# Autodesk Inventor assembly: Assembly1
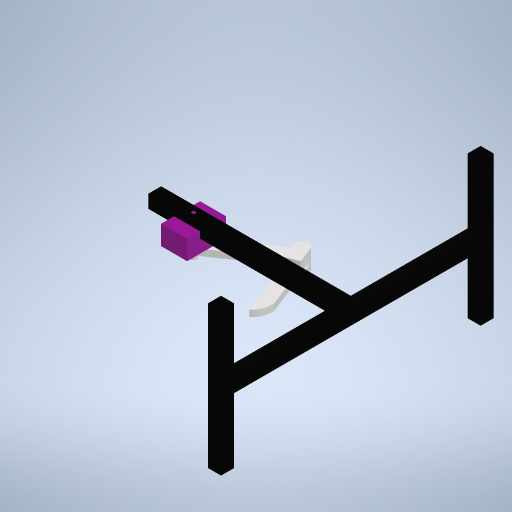
[picture p0: Inventor's stored thumbnail of the model, 512x512]
Saved by Autodesk Inventor 2024 (Build 280153000, 153)
## iProperties
Created: 2024-08-23
Part Number: Assembly1
Document SubType Name: Assembly
Designer: domko
Author: domko
## Documents named in this file (6)
- C:\Users\Public\Documents\Autodesk\Inventor 2024\czlapczlap_Leg\Assembly1.iam
- C:\Users\Public\Documents\Autodesk\Inventor 2024\czlapczlap_Leg\statyw.ipt
- C:\Users\Public\Documents\Autodesk\Inventor 2024\czlapczlap_Leg\trzymaczka.ipt
- C:\Users\Public\Documents\Autodesk\Inventor 2024\czlapczlap_Leg\arm1.ipt
- C:\Users\Public\Documents\Autodesk\Inventor 2024\czlapczlap_Leg\foot.ipt
- C:\Users\Public\Documents\Autodesk\Inventor 2024\czlapczlap_Leg\bolt.ipt
## Components (5 placed, 5 different names)
1. statyw:1 — Mate:5, Mate:6, Mate:7
2. arm1:1 — Cylindrical:1, Mate:4, Mate:10, Mate:11
3. foot:1 — Cylindrical:1, Mate:4
4. bolt:1 — Mate:8, Mate:9, Mate:11
5. trzymaczka:1 — Mate:5, Mate:6, Mate:7, Mate:8, Mate:9, Mate:10
## Relationships (9: Mate 8, CylindricalJoint 1)
- Cylindrical:1: arm1:1 ↔ foot:1
- Mate:4: arm1:1 ↔ foot:1
- Mate:5: statyw:1 ↔ trzymaczka:1
- Mate:6: statyw:1 ↔ trzymaczka:1
- Mate:7: statyw:1 ↔ trzymaczka:1
- Mate:8: bolt:1 ↔ trzymaczka:1
- Mate:9: bolt:1 ↔ trzymaczka:1
- Mate:10: arm1:1 ↔ trzymaczka:1
- Mate:11: arm1:1 ↔ bolt:1
